# Autodesk Inventor assembly: chassis_v2
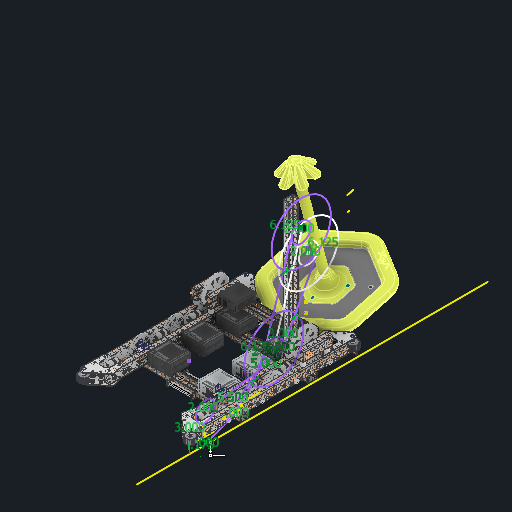
[picture p0: Inventor's stored thumbnail of the model, 512x512]
Saved by Autodesk Inventor 2025 (Build 290162000, 162)
## iProperties
Created: 2024-10-12
Part Number: chassis_v2
Document SubType Name: Assembly
Designer: Averey Ku
Author: Averey Ku
## Documents named in this file (20)
- D:\vex_robotics_high_stakes\hardware\cad\bots\high_stakes_v2\chassis_v2\chassis_v2.iam
- D:\vex_robotics_high_stakes\hardware\cad\bots\high_stakes_v2\chassis_v2\drivebay\!drivebay.iam
- D:\vex_robotics_high_stakes\hardware\cad\bots\high_stakes_v2\chassis_v2\drivebay_mirrored\!drivebay_mirrored.iam
- D:\vex_robotics_high_stakes\hardware\cad\robpros_cad_lib\Structure\C Channel\Aluminum 1x2x1\Alu C 1x2x1x23.ipt
- D:\vex_robotics_high_stakes\hardware\cad\robpros_cad_lib\Structure\Standoff\Standoff 4.00.ipt
- D:\vex_robotics_high_stakes\hardware\cad\robpros_cad_lib\Structure\Standoff.ipt
- D:\vex_robotics_high_stakes\hardware\cad\robpros_cad_lib\Motion\Spacers\Washer Steel\SWasher .375 OD x .062500.ipt
- D:\vex_robotics_high_stakes\hardware\cad\robpros_cad_lib\Motion\Spacers\Washer Steel.ipt
- C:\Users\Averey Ku\Downloads\2024-25-HighStakes-FieldCAD\276-8868-000 2024-2025 V5RC High Stakes Field\276-8868-200.iam
- D:\vex_robotics_high_stakes\hardware\cad\robpros_cad_lib\Structure\C Channel\Aluminum 1x2x1\Alu C 1x2x1x25.ipt
- D:\vex_robotics_high_stakes\hardware\cad\robpros_cad_lib\Structure\C Channel\Aluminum 1x2x1\Alu C 1x2x1x21.ipt
- D:\vex_robotics_high_stakes\hardware\cad\robpros_cad_lib\Structure\C Channel\Aluminum 1x3x1 Half Thick Cut\Alu C Half Thick 1x3x1x23.ipt
- D:\vex_robotics_high_stakes\hardware\cad\robpros_cad_lib\Motion\Spacers\Washer Steel\SWasher .375 OD x .015625.ipt
- D:\vex_robotics_high_stakes\hardware\cad\VEX-CAD-Inventor\Structure\C Channel\Aluminum 1x5x1\Alu C 1x5x1x1.ipt
- D:\vex_robotics_high_stakes\hardware\cad\VEX-CAD-Inventor\Structure\Standoff\Standoff .875.ipt
- D:\vex_robotics_high_stakes\hardware\cad\VEX-CAD-Inventor\Structure\Standoff.ipt
- D:\vex_robotics_high_stakes\hardware\cad\VEX-CAD-Inventor\Structure\Standoff\Standoff .25.ipt
- D:\vex_robotics_high_stakes\hardware\cad\VEX-CAD-Inventor\Structure\Standoff\Standoff 2.00.ipt
- D:\vex_robotics_high_stakes\hardware\cad\VEX-CAD-Inventor\Motion\Spacers\Washer Steel\SWasher .375 OD x .062500.ipt
- D:\vex_robotics_high_stakes\hardware\cad\VEX-CAD-Inventor\Motion\Spacers\Washer Steel.ipt
## Components (27 placed, 14 different names)
1. !drivebay:1 [sub-assembly] — Insert:1, Mate:1, Mate:7, Mate:9, Angle:1, Mate:10, Insert:11, Mate:11, Insert:12
2. !drivebay_mirrored:1 [sub-assembly] — Insert:2, Mate:2, Mate:3, Mate:5, Mate:12
3. Alu C 1x2x1x23:1 — Insert:1, Mate:1, Insert:2, Mate:2
4. Alu C 1x2x1x23:2 — Mate:3, Mate:5, Insert:9, Angle:2
5. Standoff 4.00:1 — Insert:6, Insert:13
6. SWasher .375 OD x .062500:1 — Insert:6
7. Standoff 4.00:2 — Insert:14
8. SWasher .375 OD x .062500:4 — Insert:9
9. 276-8868-200:1 [sub-assembly] — Mate:9, Angle:1, Angle:2, Tangent:1
10. Alu C 1x2x1x25:1
11. Alu C 1x2x1x21:1
12. Alu C 1x2x1x23:3 — Insert:11, Mate:11, Insert:15, Mate:13, Insert:16, Mate:14, Insert:17, Insert:18
13. Alu C Half Thick 1x3x1x23:1 — Insert:12, Mate:12, Tangent:1
14. SWasher .375 OD x .015625:5 — Insert:14
15. SWasher .375 OD x .015625:6 — Insert:13
16. Alu C 1x5x1x1:1 — Insert:15, Mate:13, Insert:22
17. Alu C 1x5x1x1:2 — Insert:16, Mate:14, Insert:26
18. Standoff .875:3 — Insert:17
19. Standoff .875:4 — Insert:18
20. Standoff .25:5 — Insert:19, Insert:21
21. Standoff 2.00:6 — Insert:19, Insert:20
22. SWasher .375 OD x .062500:7 — Insert:21, Insert:22
23. SWasher .375 OD x .062500:8 — Insert:20
24. Standoff .25:7
25. Standoff 2.00:8
26. SWasher .375 OD x .062500:9 — Insert:26
27. SWasher .375 OD x .062500:10
## Relationships (35: Insert 21, Mate 11, Angle 2, Tangent 1)
- Insert:1: !drivebay:1 ↔ Alu C 1x2x1x23:1
- Mate:1: !drivebay:1 ↔ Alu C 1x2x1x23:1
- Insert:2: !drivebay_mirrored:1 ↔ Alu C 1x2x1x23:1
- Mate:2: !drivebay_mirrored:1 ↔ Alu C 1x2x1x23:1
- Mate:3: !drivebay_mirrored:1 ↔ Alu C 1x2x1x23:2
- Mate:5: !drivebay_mirrored:1 ↔ Alu C 1x2x1x23:2
- Mate:7 (19.05 mm): !drivebay:1
- Insert:6: Standoff 4.00:1 ↔ SWasher .375 OD x .062500:1
- [Insert]: Standoff 4.00:2 ↔ SWasher .375 OD x .062500:4
- Insert:9: Alu C 1x2x1x23:2 ↔ SWasher .375 OD x .062500:4
- Mate:9 (-20.867 mm): !drivebay:1 ↔ 276-8868-200:1
- Angle:1 (-2 deg): !drivebay:1 ↔ 276-8868-200:1
- Angle:2 (-15 deg): Alu C 1x2x1x23:2 ↔ 276-8868-200:1
- Mate:10: !drivebay:1
- Insert:11 (15.4559 mm): !drivebay:1 ↔ Alu C 1x2x1x23:3
- Mate:11: !drivebay:1 ↔ Alu C 1x2x1x23:3
- Insert:12: !drivebay:1 ↔ Alu C Half Thick 1x3x1x23:1
- Mate:12: !drivebay_mirrored:1 ↔ Alu C Half Thick 1x3x1x23:1
- Tangent:1: 276-8868-200:1 ↔ Alu C Half Thick 1x3x1x23:1
- Insert:13: Standoff 4.00:1 ↔ SWasher .375 OD x .015625:6
- Insert:14: Standoff 4.00:2 ↔ SWasher .375 OD x .015625:5
- Insert:15: Alu C 1x2x1x23:3 ↔ Alu C 1x5x1x1:1
- Mate:13: Alu C 1x2x1x23:3 ↔ Alu C 1x5x1x1:1
- Insert:16: Alu C 1x2x1x23:3 ↔ Alu C 1x5x1x1:2
- Mate:14: Alu C 1x2x1x23:3 ↔ Alu C 1x5x1x1:2
- Insert:17: Alu C 1x2x1x23:3 ↔ Standoff .875:3
- Insert:18: Alu C 1x2x1x23:3 ↔ Standoff .875:4
- Insert:19: Standoff .25:5 ↔ Standoff 2.00:6
- Insert:20: Standoff 2.00:6 ↔ SWasher .375 OD x .062500:8
- Insert:21: Standoff .25:5 ↔ SWasher .375 OD x .062500:7
- Insert:22: Alu C 1x5x1x1:1 ↔ SWasher .375 OD x .062500:7
- [Insert]: Standoff .25:7 ↔ Standoff 2.00:8
- [Insert]: Standoff 2.00:8 ↔ SWasher .375 OD x .062500:10
- [Insert]: Standoff .25:7 ↔ SWasher .375 OD x .062500:9
- Insert:26: Alu C 1x5x1x1:2 ↔ SWasher .375 OD x .062500:9
## Named parameters: d13_d11 = 0 mm, d137_d133 = 0 mm, d138_d134 = 0 mm, d139_d135 = 0 mm
